# Autodesk Inventor assembly: linkageAssembly
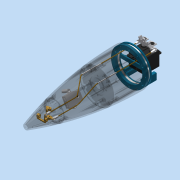
[picture p0: Inventor's stored thumbnail of the model, 180x180]
Saved by Autodesk Inventor 2017 (Build 210142000, 142)
## iProperties
Created: 2016-12-11
Part Number: linkageAssembly
Document SubType Name: Assembly
Designer: techn
Author: techn
## Documents named in this file (23)
- E:\OneDrive\Documents\Other Projects\Submarine\CAD\aft\linkageAssembly.iam
- E:\OneDrive\Documents\Other Projects\Submarine\CAD\aft\AftSectionAirtightRear.ipt
- E:\OneDrive\Documents\Other Projects\Submarine\CAD\aft\AftSectionWithSteeringLinkages.ipt
- E:\OneDrive\Documents\Other Projects\Submarine\CAD\aft\RearmostAftSection.ipt
- E:\OneDrive\Documents\Other Projects\Submarine\CAD\common\steeringYoke3mmShaft.ipt
- E:\OneDrive\Documents\Other Projects\Submarine\CAD\aft\aftSectionAirtightCap.ipt
- E:\OneDrive\Documents\Other Projects\Submarine\CAD\common\AluminumSealingDisc.ipt
- E:\OneDrive\Documents\Other Projects\Submarine\CAD\midships\AftServoSection\rearServoAttachmentPlate.ipt
- E:\OneDrive\Documents\Other Projects\Submarine\CAD\common\HitecServo\HitecServoAssembly.iam
- E:\OneDrive\Documents\Other Projects\Submarine\CAD\common\HitecServo\ServoHorn10mmPitch.ipt
- E:\OneDrive\Documents\Other Projects\Submarine\CAD\aft\planeLinkages\2mmBentFromSealDive.ipt
- E:\OneDrive\Documents\Other Projects\Submarine\CAD\aft\planeLinkages\2mmToDive.ipt
- E:\OneDrive\Documents\Other Projects\Submarine\CAD\aft\planeLinkages\2mmToSeal.ipt
- E:\OneDrive\Documents\Other Projects\Submarine\CAD\aft\planeLinkages\2mmToServo.ipt
- E:\OneDrive\Documents\Other Projects\Submarine\CAD\aft\planeLinkages\3mmHollowExpander.ipt
- E:\OneDrive\Documents\Other Projects\Submarine\CAD\aft\planeLinkages\metalClevisis.ipt
- E:\OneDrive\Documents\Other Projects\Submarine\CAD\aft\planeLinkages\2mmBentFromSealRudder.ipt
- E:\OneDrive\Documents\Other Projects\Submarine\CAD\aft\planeLinkages\2mmToRudder.ipt
- E:\OneDrive\Documents\Other Projects\Submarine\CAD\aft\planeLinkages\aftPotentiometerMount.ipt
- E:\OneDrive\Documents\Other Projects\Submarine\CAD\aft\planeLinkages\aftPotentiometers.ipt
- E:\OneDrive\Documents\Other Projects\Submarine\CAD\aft\planeLinkages\potentiometerServohornAttachment.ipt
- E:\OneDrive\Documents\Other Projects\Submarine\CAD\aft\encoder\photoTransistorAssembly.iam
- E:\OneDrive\Documents\Other Projects\Submarine\CAD\aft\encoder\photoTransistorStandoff.ipt
## Components (34 placed, 22 different names)
1. AftSectionAirtightRear:1 — Mate:1, Mate:2, Mate:5, Mate:6, Mate:45, Mate:46, Mate:101, Angle:6, Mate:105, Mate:106, Flush:3
2. AftSectionWithSteeringLinkages:1 — Mate:1, Mate:2, Mate:30, Mate:31, Mate:98, Mate:99, Mate:100
3. AluminumSealingDisc:1 — Mate:8, Mate:10, Mate:11, Mate:12, Mate:13, Mate:102
4. rearServoAttachmentPlate:1 — Mate:11, Mate:12, Mate:13, Mate:14, Mate:16, Mate:17, Mate:18, Mate:19, Mate:86, Mate:87, Mate:104
5. HitecServoAssembly:1 [sub-assembly] — Mate:14, Mate:16, Mate:20, Mate:23, Angle:3, Mate:104
6. HitecServoAssembly:2 [sub-assembly] — Mate:17, Mate:18, Mate:19, Mate:21, Mate:22, Angle:4
7. ServoHorn10mmPitch:1 — Mate:20, Mate:23, Angle:3, Mate:37
8. ServoHorn10mmPitch:2 — Mate:21, Mate:22, Mate:36, Angle:4
9. aftSectionAirtightCap:2 — Mate:5, Mate:6, Mate:8, Mate:10, Mate:101, Mate:102
10. RearmostAftSection:2 — Mate:28, Mate:29, Mate:30, Mate:31
11. steeringYoke3mmShaft:3 — Mate:29, Mate:59, Mate:60
12. steeringYoke3mmShaft:4 — Mate:28, Mate:61, Mate:77
13. metalClevisis:5 — Mate:36, Mate:71, Mate:72, Mate:91, Mate:92
14. metalClevisis:6 — Mate:37, Mate:55, Mate:56, Mate:89, Mate:93
15. 2mmToServo:7 — Mate:55, Mate:56, Ball:3
16. 2mmToSeal:4 — Mate:47, Mate:49, Ball:2
17. 2mmToSeal:5 — Mate:48, Mate:50, Ball:3
18. 3mmHollowExpander:4 — Mate:46, Mate:48, Mate:50, Mate:73, Mate:74
19. 3mmHollowExpander:5 — Mate:45, Mate:47, Mate:49, Mate:57, Mate:58
20. 2mmToDive:1 — Mate:57, Mate:58, Ball:1
21. metalClevisis:7 — Mate:59, Mate:60, Mate:69, Mate:70
22. metalClevisis:8 — Mate:61, Mate:75, Mate:76, Mate:77
23. 2mmBentFromSealDive:2 — Ball:1, Mate:69, Mate:70
24. 2mmToServo:8 — Ball:2, Mate:71, Mate:72
25. 2mmToRudder:1 — Mate:73, Mate:74, Ball:4
26. 2mmBentFromSealRudder:2 — Ball:4, Mate:75, Mate:76
27. aftPotentiometerMount:1 — Mate:84, Mate:85, Flush:1, Flush:2, Mate:86, Mate:87
28. potentiometerServohornAttachment:1 — Mate:88, Mate:89, Mate:93
29. potentiometerServohornAttachment:2 — Mate:90, Mate:91, Mate:92, Mate:103
30. aftPotentiometers:3 — Mate:85, Flush:2, Mate:88
31. aftPotentiometers:4 — Mate:84, Flush:1, Mate:90, Mate:103
32. photoTransistorAssembly:1 [sub-assembly] — Mate:94, Mate:95, Mate:96, Mate:97
33. photoTransistorStandoff:1 — Mate:94, Mate:95, Mate:99
34. photoTransistorStandoff:2 — Mate:96, Mate:97, Mate:98, Mate:100
## Relationships (81: Mate 71, BallJoint 4, Angle 3, Flush 3)
- Mate:1: AftSectionAirtightRear:1 ↔ AftSectionWithSteeringLinkages:1
- Mate:2: AftSectionAirtightRear:1 ↔ AftSectionWithSteeringLinkages:1
- Mate:5: AftSectionAirtightRear:1 ↔ aftSectionAirtightCap:2
- Mate:6: AftSectionAirtightRear:1 ↔ aftSectionAirtightCap:2
- Mate:8: AluminumSealingDisc:1 ↔ aftSectionAirtightCap:2
- Mate:10: AluminumSealingDisc:1 ↔ aftSectionAirtightCap:2
- Mate:11: AluminumSealingDisc:1 ↔ rearServoAttachmentPlate:1
- Mate:12: AluminumSealingDisc:1 ↔ rearServoAttachmentPlate:1
- Mate:13: AluminumSealingDisc:1 ↔ rearServoAttachmentPlate:1
- Mate:14: rearServoAttachmentPlate:1 ↔ HitecServoAssembly:1
- Mate:16: rearServoAttachmentPlate:1 ↔ HitecServoAssembly:1
- Mate:17: rearServoAttachmentPlate:1 ↔ HitecServoAssembly:2
- Mate:18: rearServoAttachmentPlate:1 ↔ HitecServoAssembly:2
- Mate:19: rearServoAttachmentPlate:1 ↔ HitecServoAssembly:2
- Mate:20: HitecServoAssembly:1 ↔ ServoHorn10mmPitch:1
- Mate:21: HitecServoAssembly:2 ↔ ServoHorn10mmPitch:2
- Mate:22: HitecServoAssembly:2 ↔ ServoHorn10mmPitch:2
- Mate:23: HitecServoAssembly:1 ↔ ServoHorn10mmPitch:1
- [Mate]: RearmostAftSection:2 ↔ steeringYoke3mmShaft:4
- [Mate]: RearmostAftSection:2 ↔ steeringYoke3mmShaft:3
- Mate:28 (7.747 mm): RearmostAftSection:2 ↔ steeringYoke3mmShaft:4
- Mate:29 (2.8575 mm): RearmostAftSection:2 ↔ steeringYoke3mmShaft:3
- Mate:30: AftSectionWithSteeringLinkages:1 ↔ RearmostAftSection:2
- Mate:31: AftSectionWithSteeringLinkages:1 ↔ RearmostAftSection:2
- Angle:3 (-10.982 deg): HitecServoAssembly:1 ↔ ServoHorn10mmPitch:1
- Mate:36: ServoHorn10mmPitch:2 ↔ metalClevisis:5
- Mate:37: ServoHorn10mmPitch:1 ↔ metalClevisis:6
- Mate:45: AftSectionAirtightRear:1 ↔ 3mmHollowExpander:5
- Mate:46: AftSectionAirtightRear:1 ↔ 3mmHollowExpander:4
- Mate:47: 2mmToSeal:4 ↔ 3mmHollowExpander:5
- Mate:48: 2mmToSeal:5 ↔ 3mmHollowExpander:4
- Mate:49 (-25.4 mm): 2mmToSeal:4 ↔ 3mmHollowExpander:5
- Mate:50 (-25.4 mm): 2mmToSeal:5 ↔ 3mmHollowExpander:4
- Mate:55: metalClevisis:6 ↔ 2mmToServo:7
- Mate:56: metalClevisis:6 ↔ 2mmToServo:7
- Mate:57: 3mmHollowExpander:5 ↔ 2mmToDive:1
- Mate:58 (-25.4 mm): 3mmHollowExpander:5 ↔ 2mmToDive:1
- Mate:59: steeringYoke3mmShaft:3 ↔ metalClevisis:7
- Mate:60 (0.762 mm): steeringYoke3mmShaft:3 ↔ metalClevisis:7
- Mate:61: steeringYoke3mmShaft:4 ↔ metalClevisis:8
- Ball:1: 2mmToDive:1 ↔ 2mmBentFromSealDive:2
- Mate:69: metalClevisis:7 ↔ 2mmBentFromSealDive:2
- Mate:70: metalClevisis:7 ↔ 2mmBentFromSealDive:2
- Ball:2: 2mmToSeal:4 ↔ 2mmToServo:8
- Mate:71: metalClevisis:5 ↔ 2mmToServo:8
- Mate:72: metalClevisis:5 ↔ 2mmToServo:8
- Ball:3: 2mmToServo:7 ↔ 2mmToSeal:5
- Mate:73: 3mmHollowExpander:4 ↔ 2mmToRudder:1
- Mate:74 (-25.4 mm): 3mmHollowExpander:4 ↔ 2mmToRudder:1
- Ball:4: 2mmToRudder:1 ↔ 2mmBentFromSealRudder:2
- Mate:75: metalClevisis:8 ↔ 2mmBentFromSealRudder:2
- Mate:76: metalClevisis:8 ↔ 2mmBentFromSealRudder:2
- Mate:77 (0.762 mm): steeringYoke3mmShaft:4 ↔ metalClevisis:8
- Mate:84: aftPotentiometerMount:1 ↔ aftPotentiometers:4
- Mate:85: aftPotentiometerMount:1 ↔ aftPotentiometers:3
- Flush:1: aftPotentiometerMount:1 ↔ aftPotentiometers:4
- Flush:2: aftPotentiometerMount:1 ↔ aftPotentiometers:3
- Mate:86: rearServoAttachmentPlate:1 ↔ aftPotentiometerMount:1
- Mate:87: rearServoAttachmentPlate:1 ↔ aftPotentiometerMount:1
- Mate:88: potentiometerServohornAttachment:1 ↔ aftPotentiometers:3
- Mate:89 (0.127 mm): metalClevisis:6 ↔ potentiometerServohornAttachment:1
- Mate:90: potentiometerServohornAttachment:2 ↔ aftPotentiometers:4
- Mate:91 (0.127 mm): metalClevisis:5 ↔ potentiometerServohornAttachment:2
- Mate:92: metalClevisis:5 ↔ potentiometerServohornAttachment:2
- Mate:93: metalClevisis:6 ↔ potentiometerServohornAttachment:1
- Mate:94: photoTransistorAssembly:1 ↔ photoTransistorStandoff:1
- Mate:95: photoTransistorAssembly:1 ↔ photoTransistorStandoff:1
- Mate:96: photoTransistorAssembly:1 ↔ photoTransistorStandoff:2
- Mate:97: photoTransistorAssembly:1 ↔ photoTransistorStandoff:2
- Mate:98: AftSectionWithSteeringLinkages:1 ↔ photoTransistorStandoff:2
- Mate:99: AftSectionWithSteeringLinkages:1 ↔ photoTransistorStandoff:1
- Mate:100: AftSectionWithSteeringLinkages:1 ↔ photoTransistorStandoff:2
- Mate:101: AftSectionAirtightRear:1 ↔ aftSectionAirtightCap:2
- Mate:102: AluminumSealingDisc:1 ↔ aftSectionAirtightCap:2
- Angle:4 (10 deg): HitecServoAssembly:2 ↔ ServoHorn10mmPitch:2
- Mate:103: potentiometerServohornAttachment:2 ↔ aftPotentiometers:4
- Mate:104: rearServoAttachmentPlate:1 ↔ HitecServoAssembly:1
- Angle:6 (0 deg): AftSectionAirtightRear:1
- Mate:105: AftSectionAirtightRear:1
- Mate:106: AftSectionAirtightRear:1
- Flush:3: AftSectionAirtightRear:1
## Named parameters: d30_d28 = 0 mm, d31_d29 = 0 mm
